# Autodesk Inventor assembly: cabeça_superior_4
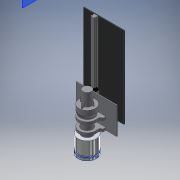
[picture p0: Inventor's stored thumbnail of the model, 180x180]
Saved by Autodesk Inventor 2018 (Build 220112000, 112)
## iProperties
Created: 2018-09-22
Part Number: cabeça_superior_4
Material: Genérico
Document SubType Name: Assembly
Designer: Usuario
Author: Usuario
## Documents named in this file (8)
- C:\Users\Usuario\Desktop\Estação BGA\Peças 3D\cabeça_superior_4.iam
- C:\Users\Usuario\Desktop\Estação BGA\Peças 3D\chapa de metal.ipt
- C:\Users\Usuario\Desktop\Estação BGA\Peças 3D\TRILHO LINEAR 15MM DFH-A_AL.ipt
- C:\Users\Usuario\Desktop\Estação BGA\Peças 3D\PATINS TRILHO LINEAR 15MM DFH-A_AL.ipt
- C:\Users\Usuario\Desktop\Estação BGA\Peças 3D\ChapaFrontalCabecaAquevimento.ipt
- C:\Users\Usuario\Desktop\Estação BGA\Peças 3D\SuporteAquecedor.ipt
- C:\Users\Usuario\Desktop\Estação BGA\Peças 3D\bocal_de_aquecimento.ipt
- C:\Users\Usuario\Desktop\Estação BGA\Peças 3D\soprador_original.ipt
## Components (8 placed, 7 different names)
1. chapa de metal:1 — Coincidência:4, Alinhamento:3, Alinhamento:4, Coincidência:12, Coincidência:13
2. TRILHO LINEAR 15MM DFH-A_AL:2 — Alinhamento:2, Coincidência:4, Alinhamento:3, Alinhamento:4
3. PATINS TRILHO LINEAR 15MM DFH-A_AL:1 — Alinhamento:2, Coincidência:5, Alinhamento:6, Alinhamento:11
4. ChapaFrontalCabecaAquevimento:1 — Coincidência:5, Alinhamento:6, Coincidência:10, Alinhamento:9, Alinhamento:11, Alinhamento:12
5. bocal_de_aquecimento:1
6. soprador_original:1 — Coincidência:11
7. SuporteAquecedor:3 — Coincidência:10, Alinhamento:9, Alinhamento:10
8. SuporteAquecedor:4 — Coincidência:11, Alinhamento:10, Alinhamento:12
## Relationships (21: Mate 12, Flush 9)
- [Mate]: TRILHO LINEAR 15MM DFH-A_AL:2 ↔ PATINS TRILHO LINEAR 15MM DFH-A_AL:1
- [Mate]: TRILHO LINEAR 15MM DFH-A_AL:2 ↔ PATINS TRILHO LINEAR 15MM DFH-A_AL:1
- Alinhamento:2 [Flush] (-0.685 mm): TRILHO LINEAR 15MM DFH-A_AL:2 ↔ PATINS TRILHO LINEAR 15MM DFH-A_AL:1
- Coincidência:4 [Mate]: chapa de metal:1 ↔ TRILHO LINEAR 15MM DFH-A_AL:2
- Alinhamento:3 [Flush]: chapa de metal:1 ↔ TRILHO LINEAR 15MM DFH-A_AL:2
- Alinhamento:4 [Flush] (40 mm): chapa de metal:1 ↔ TRILHO LINEAR 15MM DFH-A_AL:2
- Coincidência:5 [Mate]: PATINS TRILHO LINEAR 15MM DFH-A_AL:1 ↔ ChapaFrontalCabecaAquevimento:1
- Alinhamento:6 [Flush] (24 mm): PATINS TRILHO LINEAR 15MM DFH-A_AL:1 ↔ ChapaFrontalCabecaAquevimento:1
- [Mate] (25.75 mm): SuporteAquecedor:3 ↔ SuporteAquecedor:4
- [Mate]: soprador_original:1 ↔ SuporteAquecedor:3
- [Mate]: bocal_de_aquecimento:1 ↔ soprador_original:1
- [Flush] (2.5 mm): bocal_de_aquecimento:1 ↔ soprador_original:1
- [Mate] (5 mm): soprador_original:1 ↔ SuporteAquecedor:3
- Coincidência:10 [Mate]: ChapaFrontalCabecaAquevimento:1 ↔ SuporteAquecedor:3
- Alinhamento:9 [Flush] (40 mm): ChapaFrontalCabecaAquevimento:1 ↔ SuporteAquecedor:3
- Coincidência:11 [Mate]: soprador_original:1 ↔ SuporteAquecedor:4
- Alinhamento:10 [Flush]: SuporteAquecedor:3 ↔ SuporteAquecedor:4
- Coincidência:12 [Mate]: chapa de metal:1
- Coincidência:13 [Mate]: chapa de metal:1
- Alinhamento:11 [Flush]: PATINS TRILHO LINEAR 15MM DFH-A_AL:1 ↔ ChapaFrontalCabecaAquevimento:1
- Alinhamento:12 [Flush]: ChapaFrontalCabecaAquevimento:1 ↔ SuporteAquecedor:4
